# Autodesk Inventor assembly: cathode-box-on-a-flange
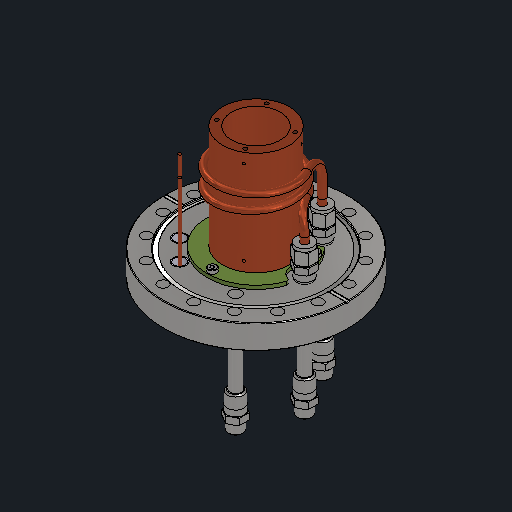
[picture p0: Inventor's stored thumbnail of the model, 512x512]
Saved by Autodesk Inventor 2026 (Build 300175050, 175E)
## iProperties
Created: 2024-05-07
Part Number: cathode-box-on-a-flange
Document SubType Name: Assembly
Designer: kuzmin
Author: kuzmin
## Documents named in this file (13)
- C:\Users\queez\Dropbox\Drawings\PIHTI\Plasma Vessel\Plasma-Flange-2024\cathode-box-on-a-flange.iam
- C:\Users\queez\Dropbox\Drawings\PIHTI\Plasma Vessel\Plasma-Flange-2024\Cathode-Flange-CF_152-70.ipt
- C:\Users\queez\Dropbox\Drawings\PIHTI\Plasma Vessel\Plasma-Flange-2024\cathode-box.ipt
- C:\Users\queez\Dropbox\Drawings\PIHTI\Plasma Vessel\Plasma-Flange-2024\cathode-box-mounting-plate.ipt
- C:\Users\queez\Dropbox\Drawings\PIHTI\Plasma Vessel\Plasma-Flange-2024\cathode-box-cooling-pipe.ipt
- C:\Users\queez\Dropbox\Drawings\PIHTI\Plasma Vessel\Plasma-Flange-2024\cathode-flange-steel-water-pipe9.3-50.ipt
- C:\Users\queez\Dropbox\Drawings\PIHTI\Plasma Vessel\Plasma-Flange-2024\SS-4-TSW-1-4.ipt
- C:\Users\queez\Dropbox\Drawings\PIHTI\Plasma Vessel\Plasma-Flange-2024\feeds\Thermocouple-Feed-D-2.1.ipt
- C:\Users\queez\Dropbox\Drawings\PIHTI\Plasma Vessel\Plasma-Flange-2024\feeds\Thermocouple-Feed-D-2.2.ipt
- C:\Users\queez\Dropbox\Drawings\PIHTI\Plasma Vessel\Plasma-Flange-2024\feeds\Electric-feed-A-6.ipt
- C:\Users\queez\Dropbox\Drawings\PIHTI\ContentCenter\Fastners\M4x8-SHCS.ipt
- C:\Users\queez\Dropbox\Drawings\PIHTI\Plasma Vessel\Plasma-Flange-2024\SS-402-1-cathode-box-flange.ipt
- C:\Users\queez\Dropbox\Drawings\PIHTI\ContentCenter\Fastners\M3x8-countersunk.ipt
## Components (25 placed, 12 different names)
1. Cathode-Flange-CF_152-70:1 — Mate:1, Mate:2, Mate:3, Mate:5, Mate:7, Rigid:1, Rotational:1, Flush:1, Mate:9, Flush:2, Flush:3, Rigid:2, Rotational:3, Rigid:3, Rotational:4
2. cathode-chamber:1 — Mate:4, Mate:5, Mate:6, Mate:12
3. cathode-box-mounting-plate:1 — Mate:1, Mate:2, Mate:3, Mate:4, Rotational:5, Rotational:6, Rigid:4, Rigid:5, Rigid:6, Rigid:7, Rigid:8, Mate:12
4. cathode-box-cooling-pipe:1 — Mate:6, Mate:7
5. cathode-flange-steel-water-pipe9.3-50:1 — Rigid:1, Mate:10, Rotational:2
6. cathode-flange-steel-water-pipe9.3-50:2 — Rotational:1, Mate:8, Cylindrical:1
7. cathode-flange-steel-water-pipe9.3-50:3 — Mate:9, Mate:11, Cylindrical:2
8. DIN 7984 M4 x 8:1 — Rotational:5
9. DIN 7984 M4 x 8:2 — Rigid:4
10. DIN 7984 M4 x 8:3 — Rotational:6
11. UNI 5933 M3 x 8:1 — Rigid:6
12. UNI 5933 M3 x 8:2 — Rigid:7
13. UNI 5933 M3 x 8:3 — Rigid:5
14. UNI 5933 M3 x 8:4 — Rigid:8
15. Thermocouple-Feed-D-2.1:1 — Rigid:2
16. Thermocouple-Feed-D-2.2:1 — Rotational:3
17. Electric-feed-A-6:1 — Rigid:3
18. Electric-feed-A-6:2 — Rotational:4
19. SS-4-TSW-1-4:1 — Mate:8, Flush:1
20. SS-4-TSW-1-4:2 — Mate:11, Flush:3, Cylindrical:2
21. SS-4-TSW-1-4:3 — Mate:10, Flush:2
22. SS-4-TSW-1-4:4 — Cylindrical:1, Rotational:7
23. SS-4-TSW-1-4:5 — Rotational:2, Rotational:8
24. SS-402-1-cathode-box-flange:1 — Rotational:8
25. SS-402-1-cathode-box-flange:2 — Rotational:7
## Relationships (33: Mate 12, WeldJoint 8, RevoluteJoint 8, Flush 3, CylindricalJoint 2)
- Mate:1: Cathode-Flange-CF_152-70:1 ↔ cathode-box-mounting-plate:1
- Mate:2: Cathode-Flange-CF_152-70:1 ↔ cathode-box-mounting-plate:1
- Mate:3: Cathode-Flange-CF_152-70:1 ↔ cathode-box-mounting-plate:1
- Mate:4: cathode-chamber:1 ↔ cathode-box-mounting-plate:1
- Mate:5: Cathode-Flange-CF_152-70:1 ↔ cathode-chamber:1
- Mate:6: cathode-chamber:1 ↔ cathode-box-cooling-pipe:1
- Mate:7: Cathode-Flange-CF_152-70:1 ↔ cathode-box-cooling-pipe:1
- Rigid:1 [WeldJoint]: Cathode-Flange-CF_152-70:1 ↔ cathode-flange-steel-water-pipe9.3-50:1
- Rotational:1 [RevoluteJoint]: Cathode-Flange-CF_152-70:1 ↔ cathode-flange-steel-water-pipe9.3-50:2
- Mate:8: cathode-flange-steel-water-pipe9.3-50:2 ↔ SS-4-TSW-1-4:1
- Flush:1 (-70 mm): Cathode-Flange-CF_152-70:1 ↔ SS-4-TSW-1-4:1
- Mate:9: Cathode-Flange-CF_152-70:1 ↔ cathode-flange-steel-water-pipe9.3-50:3
- Mate:10: cathode-flange-steel-water-pipe9.3-50:1 ↔ SS-4-TSW-1-4:3
- Flush:2 (-70 mm): Cathode-Flange-CF_152-70:1 ↔ SS-4-TSW-1-4:3
- Cylindrical:1: cathode-flange-steel-water-pipe9.3-50:2 ↔ SS-4-TSW-1-4:4
- Rotational:2 [RevoluteJoint]: cathode-flange-steel-water-pipe9.3-50:1 ↔ SS-4-TSW-1-4:5
- Mate:11: cathode-flange-steel-water-pipe9.3-50:3 ↔ SS-4-TSW-1-4:2
- Flush:3 (-70 mm): Cathode-Flange-CF_152-70:1 ↔ SS-4-TSW-1-4:2
- Cylindrical:2: cathode-flange-steel-water-pipe9.3-50:3 ↔ SS-4-TSW-1-4:2
- Rigid:2 [WeldJoint]: Cathode-Flange-CF_152-70:1 ↔ Thermocouple-Feed-D-2.1:1
- Rotational:3 [RevoluteJoint]: Cathode-Flange-CF_152-70:1 ↔ Thermocouple-Feed-D-2.2:1
- Rigid:3 [WeldJoint]: Cathode-Flange-CF_152-70:1 ↔ Electric-feed-A-6:1
- Rotational:4 [RevoluteJoint]: Cathode-Flange-CF_152-70:1 ↔ Electric-feed-A-6:2
- Rotational:5 [RevoluteJoint]: cathode-box-mounting-plate:1 ↔ DIN 7984 M4 x 8:1
- Rotational:6 [RevoluteJoint]: cathode-box-mounting-plate:1 ↔ DIN 7984 M4 x 8:3
- Rigid:4 [WeldJoint]: cathode-box-mounting-plate:1 ↔ DIN 7984 M4 x 8:2
- Rotational:7 [RevoluteJoint] (-1 mm): SS-4-TSW-1-4:4 ↔ SS-402-1-cathode-box-flange:2
- Rotational:8 [RevoluteJoint] (1 mm): SS-4-TSW-1-4:5 ↔ SS-402-1-cathode-box-flange:1
- Rigid:5 [WeldJoint]: cathode-box-mounting-plate:1 ↔ UNI 5933 M3 x 8:3
- Rigid:6 [WeldJoint]: cathode-box-mounting-plate:1 ↔ UNI 5933 M3 x 8:1
- Rigid:7 [WeldJoint]: cathode-box-mounting-plate:1 ↔ UNI 5933 M3 x 8:2
- Rigid:8 [WeldJoint]: cathode-box-mounting-plate:1 ↔ UNI 5933 M3 x 8:4
- Mate:12: cathode-chamber:1 ↔ cathode-box-mounting-plate:1
